# Autodesk Inventor assembly: First Assembly
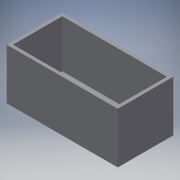
[picture p0: Inventor's stored thumbnail of the model, 180x180]
Saved by Autodesk Inventor 2018 (Build 220112000, 112)
## iProperties
Created: 2018-03-12
Part Number: First Assembly
Document SubType Name: Assembly
Designer: Josh
Author: Josh
## Documents named in this file (3)
- C:\Users\Josh\Documents\GitHub\AOS\design\First Assembly.iam
- C:\Users\Josh\Documents\GitHub\AOS\design\enclosure.ipt
- C:\Users\Josh\Documents\GitHub\AOS\design\battery.ipt
## Components (2 placed, 2 different names)
1. enclosure:1 — Mate:1, Mate:2, Mate:3
2. battery:1 — Mate:1, Mate:2, Mate:3
## Relationships (3: Mate 3)
- Mate:1: enclosure:1 ↔ battery:1
- Mate:2: enclosure:1 ↔ battery:1
- Mate:3: enclosure:1 ↔ battery:1
